# Autodesk Inventor assembly: Нога левая в сборе 2_MIR
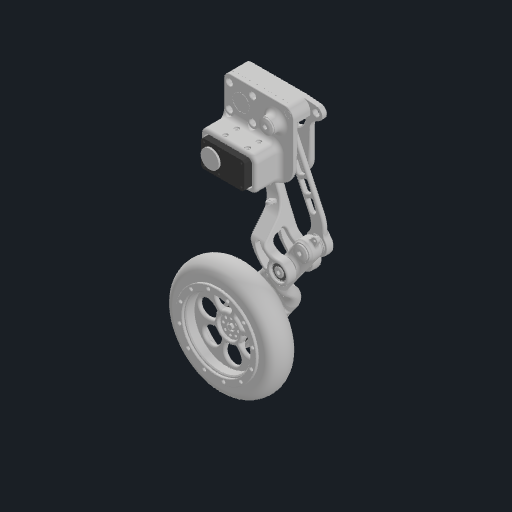
[picture p0: Inventor's stored thumbnail of the model, 512x512]
Saved by Autodesk Inventor 2025 (Build 290162010, 162A)
## iProperties
Created: 2024-06-21
Part Number: Нога левая в сборе 2_MIR
Document SubType Name: Assembly
Designer: Edward_Higgins
Author: Edward_Higgins
## Documents named in this file (12)
- D:\Users\Edward_Higgins\Desktop\ZAVOD\Робот Сколково\Нога левая в сборе 2_MIR.iam
- D:\Users\Edward_Higgins\Desktop\ZAVOD\Робот Сколково\Тяга передняя_MIR1.ipt
- D:\Users\Edward_Higgins\Desktop\ZAVOD\Робот Сколково\DYNAMIXEL XM430-W350.ipt
- D:\Users\Edward_Higgins\Desktop\ZAVOD\Робот Сколково\Голень в сборе_MIR.iam
- D:\Users\Edward_Higgins\Desktop\ZAVOD\Робот Сколково\Подшипник.ipt
- D:\Users\Edward_Higgins\Desktop\ZAVOD\Робот Сколково\Стопорная шайба.ipt
- D:\Users\Edward_Higgins\Desktop\ZAVOD\Робот Сколково\Шайба.ipt
- D:\Users\Edward_Higgins\Desktop\ZAVOD\Робот Сколково\Ось односторонняя.ipt
- D:\Users\Edward_Higgins\Desktop\ZAVOD\Робот Сколково\Колесо 2 в сборе.iam
- D:\Users\Edward_Higgins\Desktop\ZAVOD\Робот Сколково\Корпус ноги в сборе_MIR.iam
- D:\Users\Edward_Higgins\Desktop\ZAVOD\Робот Сколково\Тяга задняя 2_MIR1.ipt
- D:\Users\Edward_Higgins\Desktop\ZAVOD\Робот Сколково\Ось шарнира.ipt
## Components (12 placed, 11 different names)
1. Тяга передняя_MIR1:1 — Совмещение:84, Совмещение:21, Совмещение:85, Совмещение:82, Совмещение:103, Совмещение:115, Совмещение:114, Совмещение:113
2. DYNAMIXEL XM430-W350:1 — Совмещение:84, Совмещение:21, Совмещение:104, Угол:1
3. Голень в сборе_MIR:1 [sub-assembly] — Совмещение:85, Совмещение:82, Совмещение:100, Совмещение:99, Совмещение:106, Совмещение:105
4. Подшипник:1 — Совмещение:91, Совмещение:90, Совмещение:93, Совмещение:92, Совмещение:110
5. Стопорная шайба:1 — Совмещение:91, Совмещение:90
6. Шайба:1 — Совмещение:96, Совмещение:94, Совмещение:109, Совмещение:112
7. Ось односторонняя:1 — Совмещение:96, Совмещение:94, Совмещение:93, Совмещение:92, Совмещение:108, Совмещение:107, Совмещение:111
8. Колесо 2 в сборе:1 [sub-assembly] — Совмещение:100, Совмещение:99
9. Корпус ноги в сборе_MIR:1 [sub-assembly] — Совмещение:109, Совмещение:108, Совмещение:107, Совмещение:104, Угол:1, Совмещение:103, Совмещение:102, Совмещение:101
10. Тяга задняя 2_MIR1:1 — Совмещение:110, Совмещение:106, Совмещение:105
11. Шайба:2 — Совмещение:112, Совмещение:111
12. Ось шарнира:1 — Совмещение:115, Совмещение:114, Совмещение:113
## Relationships (28: Mate 27, Angle 1)
- Совмещение:84 [Mate]: Тяга передняя_MIR1:1 ↔ DYNAMIXEL XM430-W350:1
- Совмещение:21 [Mate]: Тяга передняя_MIR1:1 ↔ DYNAMIXEL XM430-W350:1
- Совмещение:85 [Mate]: Тяга передняя_MIR1:1 ↔ Голень в сборе_MIR:1
- Совмещение:82 [Mate]: Тяга передняя_MIR1:1 ↔ Голень в сборе_MIR:1
- Совмещение:91 [Mate]: Подшипник:1 ↔ Стопорная шайба:1
- Совмещение:90 [Mate]: Подшипник:1 ↔ Стопорная шайба:1
- Совмещение:96 [Mate]: Шайба:1 ↔ Ось односторонняя:1
- Совмещение:94 [Mate]: Шайба:1 ↔ Ось односторонняя:1
- Совмещение:93 [Mate]: Подшипник:1 ↔ Ось односторонняя:1
- Совмещение:92 [Mate]: Подшипник:1 ↔ Ось односторонняя:1
- Совмещение:100 [Mate]: Голень в сборе_MIR:1 ↔ Колесо 2 в сборе:1
- Совмещение:99 [Mate]: Голень в сборе_MIR:1 ↔ Колесо 2 в сборе:1
- Совмещение:109 [Mate]: Шайба:1 ↔ Корпус ноги в сборе_MIR:1
- Совмещение:108 [Mate]: Ось односторонняя:1 ↔ Корпус ноги в сборе_MIR:1
- Совмещение:107 [Mate]: Ось односторонняя:1 ↔ Корпус ноги в сборе_MIR:1
- Совмещение:104 [Mate]: DYNAMIXEL XM430-W350:1 ↔ Корпус ноги в сборе_MIR:1
- Угол:1 [Angle] (0 deg): DYNAMIXEL XM430-W350:1 ↔ Корпус ноги в сборе_MIR:1
- Совмещение:103 [Mate]: Тяга передняя_MIR1:1 ↔ Корпус ноги в сборе_MIR:1
- Совмещение:102 [Mate]: Корпус ноги в сборе_MIR:1
- Совмещение:101 [Mate]: Корпус ноги в сборе_MIR:1
- Совмещение:110 [Mate]: Подшипник:1 ↔ Тяга задняя 2_MIR1:1
- Совмещение:106 [Mate]: Голень в сборе_MIR:1 ↔ Тяга задняя 2_MIR1:1
- Совмещение:105 [Mate]: Голень в сборе_MIR:1 ↔ Тяга задняя 2_MIR1:1
- Совмещение:112 [Mate]: Шайба:1 ↔ Шайба:2
- Совмещение:111 [Mate]: Ось односторонняя:1 ↔ Шайба:2
- Совмещение:115 [Mate]: Тяга передняя_MIR1:1 ↔ Ось шарнира:1
- Совмещение:114 [Mate]: Тяга передняя_MIR1:1 ↔ Ось шарнира:1
- Совмещение:113 [Mate]: Тяга передняя_MIR1:1 ↔ Ось шарнира:1
